# Autodesk Inventor assembly: connection_10_19
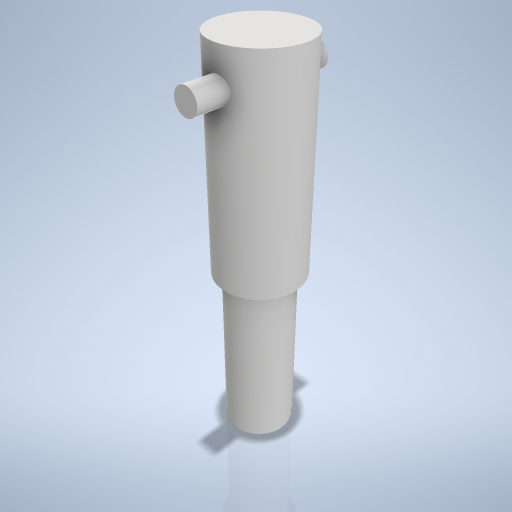
[picture p0: Inventor's stored thumbnail of the model, 512x512]
Saved by Autodesk Inventor 2024.2 (Build 282272000, 272)
## iProperties
Created: 2024-05-05
Part Number: connection_10_19
Document SubType Name: Assembly
Designer: Fabri
Author: Fabri
## Documents named in this file (3)
- C:\Users\Fabri\Documents\Inventor\stirlingEngine\connection_10_19.iam
- C:\Users\Fabri\Documents\Inventor\stirlingEngine\19.ipt
- C:\Users\Fabri\Documents\Inventor\stirlingEngine\19,1.ipt
## Components (2 placed, 2 different names)
1. 19:1 — Passend:1, Drehbar:1
2. 19,1:1 — Passend:1, Drehbar:1
## Relationships (2: Mate 1, RevoluteJoint 1)
- Passend:1 [Mate]: 19:1 ↔ 19,1:1
- Drehbar:1 [RevoluteJoint] (-44 mm): 19:1 ↔ 19,1:1
